# Autodesk Inventor assembly: leg_press_assembly
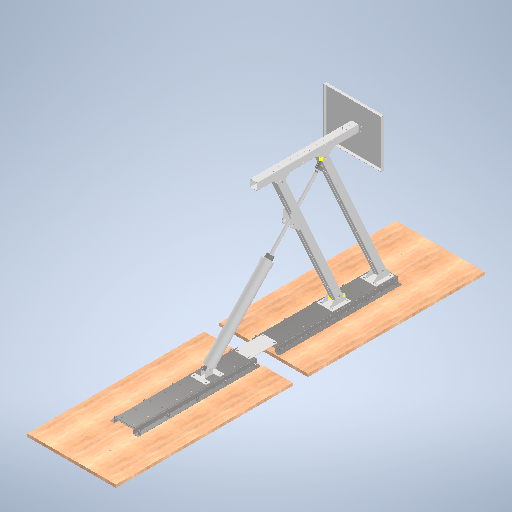
[picture p0: Inventor's stored thumbnail of the model, 512x512]
Saved by Autodesk Inventor 2025.2 (Build 292293000, 293)
## iProperties
Created: 2025-03-24
Part Number: leg_press_assembly
Document SubType Name: Assembly
Designer: Caspe
Author: Caspe
## Documents named in this file (12)
- C:\Users\Caspe\Documents\Semester 8\Project\Anomaly_Detection\Mechanical_Project\Inventor_project\leg_press_assembly.iam
- C:\Users\Caspe\Documents\Semester 8\Project\Anomaly_Detection\Mechanical_Project\Inventor_project\IMS-00-100.iam
- C:\Users\Caspe\Documents\Semester 8\Project\Anomaly_Detection\Mechanical_Project\Inventor_project\bottom_hinge.iam
- C:\Users\Caspe\Documents\Semester 8\Project\Anomaly_Detection\Mechanical_Project\Inventor_project\A1.iam
- C:\Users\Caspe\Documents\Semester 8\Project\Anomaly_Detection\Mechanical_Project\Inventor_project\B_beam.iam
- C:\Users\Caspe\Documents\Semester 8\Project\Anomaly_Detection\Mechanical_Project\Inventor_project\A_B_hinge.ipt
- C:\Users\Caspe\Documents\Semester 8\Project\Anomaly_Detection\Mechanical_Project\Inventor_project\C_plate.ipt
- C:\Users\Caspe\Documents\Semester 8\Project\Anomaly_Detection\Mechanical_Project\Inventor_project\193995 DSNU-63-500-P-A---(500PA---00--0-------0).iam
- C:\Users\Caspe\Documents\Semester 8\Project\Anomaly_Detection\Mechanical_Project\Inventor_project\Piston_floor_hinge.ipt
- C:\Users\Caspe\Documents\Semester 8\Project\Anomaly_Detection\Mechanical_Project\Inventor_project\Piston_A_beam_hinge.ipt
- C:\Users\Caspe\Documents\Semester 8\Project\Anomaly_Detection\Mechanical_Project\Inventor_project\Extender.ipt
- C:\Users\Caspe\Documents\Semester 8\Project\Anomaly_Detection\Mechanical_Project\Inventor_project\Leg_press_parameters.xlsx
## Components (17 placed, 10 different names)
1. IMS-00-100:1 [sub-assembly] — Insert:18, Insert:19, Insert:29, Insert:30, Insert:35, Insert:36
2. bottom_hinge:1 [sub-assembly] — Mate:1, Mate:2, Insert:29, Insert:30
3. A1:1 [sub-assembly] — Mate:1, Mate:2, Insert:25, Insert:26, Insert:27, Insert:28, Mate:7
4. bottom_hinge:2 [sub-assembly] — Mate:3, Mate:4, Insert:18, Insert:19
5. A1:2 [sub-assembly] — Mate:3, Mate:4, Insert:10, Insert:13
6. B_beam:1 [sub-assembly] — Insert:11, Insert:12, Insert:14, Insert:15, Insert:16, Insert:17, Insert:31, Insert:32, Insert:33, Insert:34
7. A_B_hinge:1 — Insert:31, Insert:32
8. A_B_hinge:2 — Insert:33, Insert:34, Mate:7
9. A_B_hinge:3 — Insert:13, Insert:14, Insert:15
10. A_B_hinge:4 — Insert:10, Insert:11, Insert:12
11. C_plate:1 — Insert:16, Insert:17
12. 193995 DSNU-63-500-P-A---(500PA---00--0-------0):1 [sub-assembly] — Insert:24, Mate:5, Mate:6
13. Piston_floor_hinge:1 — Insert:24, Insert:39, Insert:40
14. Piston_A_beam_hinge:1 — Insert:25, Insert:26, Mate:5
15. Piston_A_beam_hinge:2 — Insert:27, Insert:28, Mate:6
16. Extender:1 — Insert:35, Insert:36, Insert:37, Insert:38
17. IMS-00-100:2 [sub-assembly] — Insert:37, Insert:38, Insert:39, Insert:40
## Relationships (34: Insert 27, Mate 7)
- Mate:1: bottom_hinge:1 ↔ A1:1
- Mate:2 (3 mm): bottom_hinge:1 ↔ A1:1
- Mate:3: bottom_hinge:2 ↔ A1:2
- Mate:4 (3 mm): bottom_hinge:2 ↔ A1:2
- Insert:10 (2 mm): A1:2 ↔ A_B_hinge:4
- Insert:11 (2 mm): B_beam:1 ↔ A_B_hinge:4
- Insert:12 (2 mm): B_beam:1 ↔ A_B_hinge:4
- Insert:13 (2 mm): A1:2 ↔ A_B_hinge:3
- Insert:14 (2 mm): B_beam:1 ↔ A_B_hinge:3
- Insert:15 (2 mm): B_beam:1 ↔ A_B_hinge:3
- Insert:16: B_beam:1 ↔ C_plate:1
- Insert:17: B_beam:1 ↔ C_plate:1
- Insert:18: IMS-00-100:1 ↔ bottom_hinge:2
- Insert:19: IMS-00-100:1 ↔ bottom_hinge:2
- Insert:24 (3 mm): 193995 DSNU-63-500-P-A---(500PA---00--0-------0):1 ↔ Piston_floor_hinge:1
- Insert:25: A1:1 ↔ Piston_A_beam_hinge:1
- Insert:26: A1:1 ↔ Piston_A_beam_hinge:1
- Mate:5: 193995 DSNU-63-500-P-A---(500PA---00--0-------0):1 ↔ Piston_A_beam_hinge:1
- Insert:27: A1:1 ↔ Piston_A_beam_hinge:2
- Insert:28: A1:1 ↔ Piston_A_beam_hinge:2
- Mate:6: 193995 DSNU-63-500-P-A---(500PA---00--0-------0):1 ↔ Piston_A_beam_hinge:2
- Insert:29: IMS-00-100:1 ↔ bottom_hinge:1
- Insert:30: IMS-00-100:1 ↔ bottom_hinge:1
- Insert:31: B_beam:1 ↔ A_B_hinge:1
- Insert:32: B_beam:1 ↔ A_B_hinge:1
- Insert:33: B_beam:1 ↔ A_B_hinge:2
- Insert:34: B_beam:1 ↔ A_B_hinge:2
- Mate:7: A1:1 ↔ A_B_hinge:2
- Insert:35: IMS-00-100:1 ↔ Extender:1
- Insert:36: IMS-00-100:1 ↔ Extender:1
- Insert:37: Extender:1 ↔ IMS-00-100:2
- Insert:38: Extender:1 ↔ IMS-00-100:2
- Insert:39: Piston_floor_hinge:1 ↔ IMS-00-100:2
- Insert:40: Piston_floor_hinge:1 ↔ IMS-00-100:2
## Named parameters: A_length = 1000 mm, A_width = 50 mm, A_bend = 20 mm, A_connection_width = 40 mm, A_displacement = 500 mm, A_hole_height = 10 mm, A_hole_length = 40 mm, A_joint_diameter = 16 mm, A_height = 50 mm, A_joint_tolerance = 3 mm, l___________ = 0 mm, B_length = 700 mm, B_width = 50 mm, B_bend = 20 mm, B_connection_width = 40 mm, B_hole_height = 10 mm, B_hole_length = 40 mm, l__________ = 0 mm, C_length = 400 mm, C_width = 20 mm, C_height = 330 mm, l_________ = 0 mm, rivet_diameter = 3.35 mm, rivet_displacement = 250 mm, plate_thickness = 1.5 mm, l________ = 0 mm, B_hinge_holes_spacing = 50 mm, B_height = 50 mm, A_B_spacing = 2 mm, L_Piston_Bottom = 21 mm, L_Piston_Top = 25 mm
